# Autodesk Inventor assembly: CHAIN
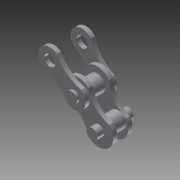
[picture p0: Inventor's stored thumbnail of the model, 180x180]
Saved by Autodesk Inventor 2011 (Build 150239000, 239)
## iProperties
Created: 2013-01-14
Part Number: CHAIN
Document SubType Name: Assembly
Designer: 971065
Author: 971065
## Documents named in this file (4)
- C:\Users\Danny\Documents\GitHub\2013CAD\2013 robot\Spiderbot\CHAIN.iam
- C:\Users\Danny\Documents\GitHub\2013CAD\2013 robot\Common assemblies\Chain Parts\chain_axel.ipt
- C:\Users\Danny\Documents\GitHub\2013CAD\2013 robot\Common assemblies\Chain Parts\inner_link.ipt
- C:\Users\Danny\Documents\GitHub\2013CAD\2013 robot\Common assemblies\Chain Parts\outter_link.ipt
## Components (6 placed, 3 different names)
1. chain_axel:3 — Insert:1, Insert:2, Insert:3
2. inner_link:11 — Insert:2, Mate:1, Mate:2
3. inner_link:13 — Insert:1, Insert:4
4. outter_link:6 — Insert:3
5. outter_link:7 — Insert:4
6. chain_axel:4 — Mate:1, Mate:2
## Relationships (6: Insert 4, Mate 2)
- Insert:1 (-3.302 mm): chain_axel:3 ↔ inner_link:13
- Insert:2 (-3.302 mm): chain_axel:3 ↔ inner_link:11
- Insert:3 (-0.762 mm): chain_axel:3 ↔ outter_link:6
- Insert:4 (-1.27 mm): inner_link:13 ↔ outter_link:7
- Mate:1: inner_link:11 ↔ chain_axel:4
- Mate:2: inner_link:11 ↔ chain_axel:4
